# Autodesk Inventor assembly: ps3_eye_assembly2
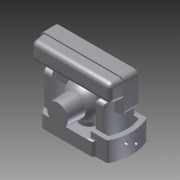
[picture p0: Inventor's stored thumbnail of the model, 180x180]
Saved by Autodesk Inventor 2011 (Build 150239000, 239)
## iProperties
Created: 2010-06-24
Part Number: ps3_eye_assembly2
Document SubType Name: Assembly
Designer: abarry
Author: abarry
## Documents named in this file (3)
- C:\Documents and Settings\abarry\My Documents\CAD\ps3_eye_assembly2.iam
- C:\Documents and Settings\abarry\My Documents\CAD\ps3_eye.ipt
- C:\Documents and Settings\abarry\My Documents\CAD\PS3_eye_holder_from_base.ipt
## Components (2 placed, 2 different names)
1. ps3_eye:1 — Flush:1, Mate:1, Mate:2
2. PS3_eye_holder_from_base:1 — Flush:1, Mate:1, Mate:2
## Relationships (3: Mate 2, Flush 1)
- Flush:1: ps3_eye:1 ↔ PS3_eye_holder_from_base:1
- Mate:1: ps3_eye:1 ↔ PS3_eye_holder_from_base:1
- Mate:2: ps3_eye:1 ↔ PS3_eye_holder_from_base:1
